# Autodesk Inventor assembly: forcefoot
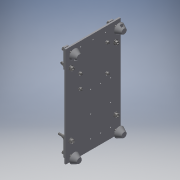
[picture p0: Inventor's stored thumbnail of the model, 180x180]
Saved by Autodesk Inventor 2018 (Build 220112000, 112)
## iProperties
Created: 2018-12-03
Part Number: forcefoot
Document SubType Name: Assembly
Designer: jaspe
Author: jaspe
## Documents named in this file (14)
- C:\Users\jaspe\bitbots_hardware\wolfgang\assembly\legs\foot\forcefoot.iam
- C:\Users\jaspe\bitbots_hardware\wolfgang\assembly\legs\foot\load_cell.ipt
- C:\Users\jaspe\bitbots_hardware\wolfgang\assembly\legs\foot.ipt
- C:\Users\jaspe\Documents\Inventor\Content Center Files\R2018\en-US\DIN EN ISO 4032\DIN EN ISO 4032 - M4.ipt
- C:\Users\jaspe\bitbots_hardware\wolfgang\stollen_m4.ipt
- C:\Users\jaspe\Documents\Inventor\Content Center Files\R2018\en-US\DIN EN ISO 7089\DIN EN ISO 7089 -  4.ipt
- C:\Users\jaspe\Documents\Inventor\Content Center Files\R2018\en-US\ISO 10511\ISO 10511 - M4.ipt
- C:\Users\jaspe\Documents\Inventor\Content Center Files\R2018\en-US\ISO 4762(2)\ISO 4762 - M4 x 25ISO.ipt
- C:\Users\jaspe\bitbots_hardware\wolfgang\assembly\legs\foot\pcb_assembly.iam
- C:\Users\jaspe\Documents\Inventor\Content Center Files\R2018\en-US\ISO 10511\ISO 10511 - M3.ipt
- C:\Users\jaspe\Documents\Inventor\Content Center Files\R2018\en-US\DIN EN ISO 4032\DIN EN ISO 4032 - M3.ipt
- C:\Users\jaspe\Documents\Inventor\Content Center Files\R2018\en-US\ISO 4762(2)\ISO 4762 - M3 x 12ISO.ipt
- C:\Users\jaspe\Documents\Inventor\Content Center Files\R2018\en-US\ISO 4762(2)\ISO 4762 - M4 x 20ISO.ipt
- C:\Users\jaspe\bitbots_hardware\wolfgang\assembly\legs\foot\foot_cover.ipt
## Components (55 placed, 13 different names)
1. foot:1 — Mate:1, Mate:2, Mate:22, Mate:34, Mate:53, Mate:54, Mate:55, Mate:56, Mate:91, Mate:92, Mate:93, Mate:94, Mate:95, Mate:96, Mate:97, Mate:98, Mate:101, Mate:102, Mate:104, Mate:105, Mate:112, Mate:113, Mate:115, Mate:117, Mate:123, Mate:126, Mate:129, Mate:130, Mate:131
2. load_cell:1 — Mate:1, Mate:2, Mate:17, Mate:18, Mate:19, Mate:20, Mate:23, Mate:25, Mate:26, Mate:27, Mate:28, Mate:29, Mate:30, Mate:32, Mate:33
3. ISO 4762 M4 x 25:2 — Mate:32, Mate:35, Mate:128
4. DIN EN ISO 7089 4:4 — Mate:33, Mate:34, Mate:35
5. DIN EN ISO 7089 4:2 — Mate:22, Mate:23, Mate:24
6. DIN EN ISO 4032 M4:2 — Mate:20, Mate:21, Mate:24
7. DIN EN ISO 7089 4:1 — Mate:18, Mate:19, Mate:21
8. DIN EN ISO 10511 M4:1 — Mate:25, Mate:26
9. ISO 4762 M4 x 25:1 — Mate:27, Mate:28, Mate:31
10. DIN EN ISO 4032 M4:4 — Mate:17, Mate:29
11. stollen_m4:1 — Mate:30, Mate:31
12. load_cell:2
13. DIN EN ISO 4032 M4:5
14. stollen_m4:2
15. DIN EN ISO 4032 M4:6
16. DIN EN ISO 7089 4:5
17. ISO 4762 M4 x 20:1 — Mate:54
18. DIN EN ISO 10511 M4:2
19. ISO 4762 M4 x 25:4 — Mate:53
20. DIN EN ISO 7089 4:6 — Mate:56
21. DIN EN ISO 7089 4:7 — Mate:55
22. load_cell:3
23. DIN EN ISO 4032 M4:7
24. stollen_m4:3
25. DIN EN ISO 4032 M4:8
26. DIN EN ISO 7089 4:8
27. ISO 4762 M4 x 25:5 — Mate:96, Mate:127
28. DIN EN ISO 10511 M4:3
29. ISO 4762 M4 x 25:6 — Mate:95
30. DIN EN ISO 7089 4:9 — Mate:98
31. DIN EN ISO 7089 4:10 — Mate:97
32. load_cell:4
33. DIN EN ISO 4032 M4:9
34. stollen_m4:4
35. DIN EN ISO 4032 M4:10
36. DIN EN ISO 7089 4:11
37. ISO 4762 M4 x 20:2 — Mate:91
38. DIN EN ISO 10511 M4:4
39. ISO 4762 M4 x 25:8 — Mate:92
40. DIN EN ISO 7089 4:12 — Mate:93
41. DIN EN ISO 7089 4:13 — Mate:94
42. pcb_assembly:1 [sub-assembly] — Mate:99, Mate:100, Mate:103, Mate:111, Mate:116, Mate:118, Mate:119, Mate:121, Mate:124, Mate:125
43. DIN EN ISO 10511 M3:1 — Mate:105, Mate:106
44. ISO 4762 M3 x 12:1 — Mate:99, Mate:100, Mate:101, Mate:106
45. DIN EN ISO 4032 M3:1 — Mate:102, Mate:103, Mate:104
46. DIN EN ISO 10511 M3:2 — Mate:117
47. ISO 4762 M3 x 12:2 — Mate:116, Mate:118, Mate:120
48. DIN EN ISO 4032 M3:2 — Mate:120, Mate:121
49. DIN EN ISO 10511 M3:3 — Mate:126
50. ISO 4762 M3 x 12:3 — Mate:122, Mate:124, Mate:125
51. DIN EN ISO 4032 M3:3 — Mate:122, Mate:123
52. DIN EN ISO 10511 M3:5 — Mate:113
53. ISO 4762 M3 x 12:5 — Mate:111, Mate:112, Mate:114, Mate:119
54. DIN EN ISO 4032 M3:5 — Mate:114, Mate:115
55. foot_cover:1 — Mate:127, Mate:128, Mate:129
## Relationships (116: Mate 116)
- Mate:1: foot:1 ↔ load_cell:1
- Mate:2: foot:1 ↔ load_cell:1
- Mate:17: load_cell:1 ↔ DIN EN ISO 4032 M4:4
- Mate:18: load_cell:1 ↔ DIN EN ISO 7089 4:1
- Mate:19: load_cell:1 ↔ DIN EN ISO 7089 4:1
- Mate:20: load_cell:1 ↔ DIN EN ISO 4032 M4:2
- Mate:21: DIN EN ISO 4032 M4:2 ↔ DIN EN ISO 7089 4:1
- Mate:22: foot:1 ↔ DIN EN ISO 7089 4:2
- Mate:23: load_cell:1 ↔ DIN EN ISO 7089 4:2
- Mate:24: DIN EN ISO 7089 4:2 ↔ DIN EN ISO 4032 M4:2
- Mate:25: load_cell:1 ↔ DIN EN ISO 10511 M4:1
- Mate:26: load_cell:1 ↔ DIN EN ISO 10511 M4:1
- Mate:27: load_cell:1 ↔ ISO 4762 M4 x 25:1
- Mate:28: load_cell:1 ↔ ISO 4762 M4 x 25:1
- Mate:29: load_cell:1 ↔ DIN EN ISO 4032 M4:4
- Mate:30: load_cell:1 ↔ stollen_m4:1
- Mate:31: ISO 4762 M4 x 25:1 ↔ stollen_m4:1
- Mate:32: load_cell:1 ↔ ISO 4762 M4 x 25:2
- Mate:33: load_cell:1 ↔ DIN EN ISO 7089 4:4
- Mate:34: foot:1 ↔ DIN EN ISO 7089 4:4
- Mate:35: ISO 4762 M4 x 25:2 ↔ DIN EN ISO 7089 4:4
- [Mate]: load_cell:2 ↔ DIN EN ISO 4032 M4:6
- [Mate]: load_cell:2 ↔ DIN EN ISO 7089 4:5
- [Mate]: load_cell:2 ↔ DIN EN ISO 7089 4:5
- [Mate]: load_cell:2 ↔ DIN EN ISO 4032 M4:5
- [Mate]: DIN EN ISO 4032 M4:5 ↔ DIN EN ISO 7089 4:5
- [Mate]: load_cell:2 ↔ DIN EN ISO 7089 4:6
- [Mate]: DIN EN ISO 4032 M4:5 ↔ DIN EN ISO 7089 4:6
- [Mate]: load_cell:2 ↔ DIN EN ISO 10511 M4:2
- [Mate]: load_cell:2 ↔ DIN EN ISO 10511 M4:2
- [Mate]: load_cell:2 ↔ ISO 4762 M4 x 25:4
- [Mate]: load_cell:2 ↔ ISO 4762 M4 x 25:4
- [Mate]: load_cell:2 ↔ DIN EN ISO 4032 M4:6
- [Mate]: load_cell:2 ↔ stollen_m4:2
- [Mate]: stollen_m4:2 ↔ ISO 4762 M4 x 25:4
- [Mate]: load_cell:2 ↔ ISO 4762 M4 x 20:1
- [Mate]: load_cell:2 ↔ DIN EN ISO 7089 4:7
- [Mate]: ISO 4762 M4 x 20:1 ↔ DIN EN ISO 7089 4:7
- Mate:53: foot:1 ↔ ISO 4762 M4 x 25:4
- Mate:54: foot:1 ↔ ISO 4762 M4 x 20:1
- Mate:55: foot:1 ↔ DIN EN ISO 7089 4:7
- Mate:56: foot:1 ↔ DIN EN ISO 7089 4:6
- [Mate]: load_cell:3 ↔ DIN EN ISO 4032 M4:8
- [Mate]: load_cell:3 ↔ DIN EN ISO 7089 4:8
- [Mate]: load_cell:3 ↔ DIN EN ISO 7089 4:8
- [Mate]: load_cell:3 ↔ DIN EN ISO 4032 M4:7
- [Mate]: DIN EN ISO 4032 M4:7 ↔ DIN EN ISO 7089 4:8
- [Mate]: load_cell:3 ↔ DIN EN ISO 7089 4:9
- [Mate]: DIN EN ISO 4032 M4:7 ↔ DIN EN ISO 7089 4:9
- [Mate]: load_cell:3 ↔ DIN EN ISO 10511 M4:3
- [Mate]: load_cell:3 ↔ DIN EN ISO 10511 M4:3
- [Mate]: load_cell:3 ↔ ISO 4762 M4 x 25:6
- [Mate]: load_cell:3 ↔ ISO 4762 M4 x 25:6
- [Mate]: load_cell:3 ↔ DIN EN ISO 4032 M4:8
- [Mate]: load_cell:3 ↔ stollen_m4:3
- [Mate]: stollen_m4:3 ↔ ISO 4762 M4 x 25:6
- [Mate]: load_cell:3 ↔ ISO 4762 M4 x 25:5
- [Mate]: load_cell:3 ↔ DIN EN ISO 7089 4:10
- [Mate]: ISO 4762 M4 x 25:5 ↔ DIN EN ISO 7089 4:10
- [Mate]: load_cell:4 ↔ DIN EN ISO 4032 M4:10
- [Mate]: load_cell:4 ↔ DIN EN ISO 7089 4:11
- [Mate]: load_cell:4 ↔ DIN EN ISO 7089 4:11
- [Mate]: load_cell:4 ↔ DIN EN ISO 4032 M4:9
- [Mate]: DIN EN ISO 4032 M4:9 ↔ DIN EN ISO 7089 4:11
- [Mate]: load_cell:4 ↔ DIN EN ISO 7089 4:12
- [Mate]: DIN EN ISO 4032 M4:9 ↔ DIN EN ISO 7089 4:12
- [Mate]: load_cell:4 ↔ DIN EN ISO 10511 M4:4
- [Mate]: load_cell:4 ↔ DIN EN ISO 10511 M4:4
- [Mate]: load_cell:4 ↔ ISO 4762 M4 x 25:8
- [Mate]: load_cell:4 ↔ ISO 4762 M4 x 25:8
- [Mate]: load_cell:4 ↔ DIN EN ISO 4032 M4:10
- [Mate]: load_cell:4 ↔ stollen_m4:4
- [Mate]: stollen_m4:4 ↔ ISO 4762 M4 x 25:8
- [Mate]: load_cell:4 ↔ ISO 4762 M4 x 20:2
- [Mate]: load_cell:4 ↔ DIN EN ISO 7089 4:13
- [Mate]: ISO 4762 M4 x 20:2 ↔ DIN EN ISO 7089 4:13
- Mate:91: foot:1 ↔ ISO 4762 M4 x 20:2
- Mate:92: foot:1 ↔ ISO 4762 M4 x 25:8
- Mate:93: foot:1 ↔ DIN EN ISO 7089 4:12
- Mate:94: foot:1 ↔ DIN EN ISO 7089 4:13
- Mate:95: foot:1 ↔ ISO 4762 M4 x 25:6
- Mate:96: foot:1 ↔ ISO 4762 M4 x 25:5
- Mate:97: foot:1 ↔ DIN EN ISO 7089 4:10
- Mate:98: foot:1 ↔ DIN EN ISO 7089 4:9
- Mate:99: pcb_assembly:1 ↔ ISO 4762 M3 x 12:1
- Mate:100: pcb_assembly:1 ↔ ISO 4762 M3 x 12:1
- Mate:101: foot:1 ↔ ISO 4762 M3 x 12:1
- Mate:102: foot:1 ↔ DIN EN ISO 4032 M3:1
- Mate:103: pcb_assembly:1 ↔ DIN EN ISO 4032 M3:1
- Mate:104: foot:1 ↔ DIN EN ISO 4032 M3:1
- Mate:105: foot:1 ↔ DIN EN ISO 10511 M3:1
- Mate:106: DIN EN ISO 10511 M3:1 ↔ ISO 4762 M3 x 12:1
- [Mate]: DIN EN ISO 10511 M3:2 ↔ ISO 4762 M3 x 12:2
- [Mate]: DIN EN ISO 10511 M3:3 ↔ ISO 4762 M3 x 12:3
- [Mate]: DIN EN ISO 10511 M3:5 ↔ ISO 4762 M3 x 12:5
- Mate:111: pcb_assembly:1 ↔ ISO 4762 M3 x 12:5
- Mate:112: foot:1 ↔ ISO 4762 M3 x 12:5
- Mate:113: foot:1 ↔ DIN EN ISO 10511 M3:5
- Mate:114: ISO 4762 M3 x 12:5 ↔ DIN EN ISO 4032 M3:5
- Mate:115: foot:1 ↔ DIN EN ISO 4032 M3:5
- Mate:116: pcb_assembly:1 ↔ ISO 4762 M3 x 12:2
- Mate:117: foot:1 ↔ DIN EN ISO 10511 M3:2
- Mate:118: pcb_assembly:1 ↔ ISO 4762 M3 x 12:2
- Mate:119: pcb_assembly:1 ↔ ISO 4762 M3 x 12:5
- Mate:120: ISO 4762 M3 x 12:2 ↔ DIN EN ISO 4032 M3:2
- Mate:121: pcb_assembly:1 ↔ DIN EN ISO 4032 M3:2
- Mate:122: ISO 4762 M3 x 12:3 ↔ DIN EN ISO 4032 M3:3
- Mate:123: foot:1 ↔ DIN EN ISO 4032 M3:3
- Mate:124: pcb_assembly:1 ↔ ISO 4762 M3 x 12:3
- Mate:125: pcb_assembly:1 ↔ ISO 4762 M3 x 12:3
- Mate:126: foot:1 ↔ DIN EN ISO 10511 M3:3
- Mate:127: ISO 4762 M4 x 25:5 ↔ foot_cover:1
- Mate:128: ISO 4762 M4 x 25:2 ↔ foot_cover:1
- Mate:129: foot:1 ↔ foot_cover:1
- Mate:130: foot:1
- Mate:131: foot:1
## Named parameters: d53_d52 = 0 mm, d54_d39 = 0 mm, d55_d40 = 0 mm, d56_d41 = 0 mm, d57_d42 = 0 mm, d58_d43 = 0 mm, d59_d44 = 0 mm, d60_d45 = 0 mm, d61_d46 = 0 mm, d62_d47 = 0 mm, d63_d48 = 0 mm, d64_d50 = 0 mm, d65_d20 = 0 mm, d66_d34 = 0 mm, d67_d35 = 0 mm, d68_d36 = 0 mm, d69_d37 = 0 mm, d74_d52 = 0 mm, d75_d39 = 0 mm, d76_d40 = 0 mm, d77_d41 = 0 mm, d78_d42 = 0 mm, d79_d43 = 0 mm, d80_d44 = 0 mm, d81_d45 = 0 mm, d82_d46 = 0 mm, d83_d47 = 0 mm, d84_d48 = 0 mm, d85_d50 = 0 mm, d86_d20 = 0 mm, d87_d34 = 0 mm, d88_d35 = 0 mm, d89_d36 = 0 mm, d90_d37 = 0 mm, d91_d52 = 0 mm, d92_d39 = 0 mm, d93_d40 = 0 mm, d94_d41 = 0 mm, d95_d42 = 0 mm, d96_d43 = 0 mm, d97_d44 = 0 mm, d98_d45 = 0 mm, d99_d46 = 0 mm, d100_d47 = 0 mm, d101_d48 = 0 mm, d102_d50 = 0 mm, d103_d20 = 0 mm, d104_d34 = 0 mm, d105_d35 = 0 mm, d106_d36 = 0 mm, d107_d37 = 0 mm, d127_d126 = 0 mm, d128_d126 = 0 mm, d130_d126 = 0 mm
